# Autodesk Inventor assembly: font arm
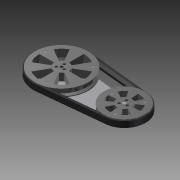
[picture p0: Inventor's stored thumbnail of the model, 180x180]
Saved by Autodesk Inventor 2011 (Build 150239000, 239)
## iProperties
Created: 2010-04-19
Part Number: font arm
Document SubType Name: Assembly
Designer: lucio
Mass: 643.177 g
Surface Area: 2107.64 cm^2
Volume: 655.52 cm^3
Density: 0.981169 g/cm^3
Author: lucio
## Documents named in this file (6)
- C:\Users\lucio\Documents\Inventor\caterpillar\font arm.iam
- C:\Users\lucio\Documents\Inventor\caterpillar\short arm.ipt
- C:\Users\lucio\Documents\Inventor\caterpillar\small base wheel.iam
- C:\Users\lucio\Documents\Inventor\caterpillar\short axle.ipt
- C:\Users\lucio\Documents\Inventor\caterpillar\small belt.ipt
- C:\Users\lucio\Documents\Inventor\caterpillar\base wheel.iam
## Components (5 placed, 5 different names)
1. short arm:1 — Flush:1, Mate:1, Mate:3, Mate:4, Mate:5
2. small base wheel:1 [sub-assembly] — Mate:2, Mate:5, Mate:6
3. short axle:1 — Flush:1, Mate:1, Mate:2
4. small belt:1 — Flush:2, Mate:6, Mate:7
5. base wheel:1 [sub-assembly] — Mate:3, Flush:2, Mate:4, Mate:7
## Relationships (9: Mate 7, Flush 2)
- Flush:1: short arm:1 ↔ short axle:1
- Mate:1: short arm:1 ↔ short axle:1
- Mate:2: small base wheel:1 ↔ short axle:1
- Mate:3: short arm:1 ↔ base wheel:1
- Flush:2 (2 mm): small belt:1 ↔ base wheel:1
- Mate:4 (2 mm): short arm:1 ↔ base wheel:1
- Mate:5 (2 mm): short arm:1 ↔ small base wheel:1
- Mate:6: small base wheel:1 ↔ small belt:1
- Mate:7: small belt:1 ↔ base wheel:1
